# Autodesk Inventor assembly: Foot
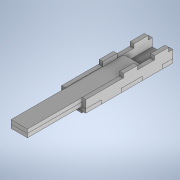
[picture p0: Inventor's stored thumbnail of the model, 180x180]
Saved by Autodesk Inventor 2020 (Build 240168000, 168)
## iProperties
Created: 2019-12-19
Part Number: Foot
Document SubType Name: Assembly
Designer: damien
Author: damien
## Documents named in this file (5)
- D:\fablab\sawbench\Foot.iam
- D:\fablab\sawbench\graduated_foot_03.ipt
- D:\fablab\sawbench\rail.ipt
- D:\fablab\sawbench\cover.ipt
- D:\fablab\sawbench\nut_blocker.ipt
## Components (6 placed, 4 different names)
1. graduated_foot_03:1 — Placage:1, Affleurement:1, Affleurement:2, Affleurement:3, Affleurement:4, Affleurement:5, Affleurement:6, Placage:13
2. graduated_foot_03:2 — Placage:1, Affleurement:1, Affleurement:2, Affleurement:3, Placage:12, Affleurement:15
3. rail:1 — Placage:13, Affleurement:11, Affleurement:12, Affleurement:13, Affleurement:14, Placage:14, Affleurement:15, Placage:15, Affleurement:16, Affleurement:17
4. cover:1 — Affleurement:10, Placage:12, Affleurement:11, Affleurement:14, Placage:14
5. cover:2 — Affleurement:10, Affleurement:12, Affleurement:13
6. nut_blocker:1 — Placage:15, Affleurement:16, Affleurement:17
## Relationships (19: Flush 14, Mate 5)
- Placage:1 [Mate]: graduated_foot_03:1 ↔ graduated_foot_03:2
- Affleurement:1 [Flush]: graduated_foot_03:1 ↔ graduated_foot_03:2
- Affleurement:2 [Flush]: graduated_foot_03:1 ↔ graduated_foot_03:2
- Affleurement:3 [Flush]: graduated_foot_03:1 ↔ graduated_foot_03:2
- Affleurement:4 [Flush]: graduated_foot_03:1
- Affleurement:5 [Flush]: graduated_foot_03:1
- Affleurement:6 [Flush]: graduated_foot_03:1
- Affleurement:10 [Flush]: cover:1 ↔ cover:2
- Placage:12 [Mate]: graduated_foot_03:2 ↔ cover:1
- Placage:13 [Mate]: graduated_foot_03:1 ↔ rail:1
- Affleurement:11 [Flush]: rail:1 ↔ cover:1
- Affleurement:12 [Flush]: rail:1 ↔ cover:2
- Affleurement:13 [Flush]: rail:1 ↔ cover:2
- Affleurement:14 [Flush]: rail:1 ↔ cover:1
- Placage:14 [Mate]: rail:1 ↔ cover:1
- Affleurement:15 [Flush] (140 mm): graduated_foot_03:2 ↔ rail:1
- Placage:15 [Mate]: rail:1 ↔ nut_blocker:1
- Affleurement:16 [Flush] (29 mm): rail:1 ↔ nut_blocker:1
- Affleurement:17 [Flush] (10 mm): rail:1 ↔ nut_blocker:1
